# Autodesk Inventor assembly: Ganymede Node
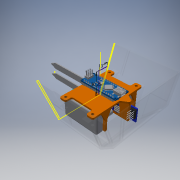
[picture p0: Inventor's stored thumbnail of the model, 180x180]
Saved by Autodesk Inventor 2017 (Build 210142000, 142)
## iProperties
Created: 2017-04-29
Part Number: Ganymede Node
Document SubType Name: Assembly
Designer: X220T
Author: X220T
## Documents named in this file (11)
- C:\Google Drive\Projects\Hackathon\RenoSpaceApps2017\Node Components\Ganymede Node.iam
- C:\Google Drive\Projects\Hackathon\RenoSpaceApps2017\Node Components\NanoV3 v4.ipt
- C:\Google Drive\Projects\Hackathon\RenoSpaceApps2017\Node Components\NRF24L01+.ipt
- C:\Google Drive\Projects\Hackathon\RenoSpaceApps2017\Node Components\solar cell 26x52.ipt
- C:\Google Drive\Projects\Hackathon\RenoSpaceApps2017\Node Components\soil sensor.ipt
- C:\Google Drive\Projects\Hackathon\RenoSpaceApps2017\Node Components\moist probe.ipt
- C:\Google Drive\Projects\Hackathon\RenoSpaceApps2017\Node Components\core printed.ipt
- C:\Google Drive\Projects\Hackathon\RenoSpaceApps2017\Node Components\Step Down voltage regulator LM2596.ipt
- C:\Google Drive\Projects\Hackathon\RenoSpaceApps2017\Node Components\battery.ipt
- C:\Google Drive\Projects\Hackathon\RenoSpaceApps2017\Node Components\Case 1.ipt
- C:\Google Drive\Projects\Hackathon\RenoSpaceApps2017\Node Components\Case 2.ipt
## Components (16 placed, 10 different names)
1. NanoV3 v4:1 — Mate:2, Mate:3, Flush:5
2. NRF24L01+:1 — Mate:6, Flush:6, Mate:7
3. soil sensor:1 — Mate:1, Flush:1, Flush:2
4. moist probe:1 — Mate:1, Flush:1, Flush:2, Flush:3, Mate:2, Mate:3, Mate:4, Flush:4, Mate:5, Flush:5, Mate:6, Flush:6, Mate:7
5. core printed:1 — Flush:3, Rotational:1, Flush:7
6. Step Down voltage regulator LM2596:1 — Rotational:1
7. battery:1
8. battery:2
9. Case 1:1 — Planar:1, Planar:2, Planar:3, Planar:4, Planar:6, Flush:7, Flush:8, Flush:9
10. solar cell 26x52:7
11. solar cell 26x52:9 — Planar:6
12. solar cell 26x52:11 — Planar:3
13. solar cell 26x52:13 — Planar:4
14. solar cell 26x52:15 — Planar:1
15. solar cell 26x52:16 — Planar:2
16. Case 2:1 — Flush:8, Flush:9
## Relationships (22: Flush 9, Mate 7, PlanarJoint 5, RevoluteJoint 1)
- Mate:1 (3.95 mm): soil sensor:1 ↔ moist probe:1
- Flush:1 (-2.68 mm): soil sensor:1 ↔ moist probe:1
- Flush:2: soil sensor:1 ↔ moist probe:1
- Flush:3: moist probe:1 ↔ core printed:1
- Mate:2 (4 mm): NanoV3 v4:1 ↔ moist probe:1
- Mate:3 (-4 mm): NanoV3 v4:1 ↔ moist probe:1
- Mate:4: moist probe:1
- Flush:4: moist probe:1
- Mate:5: moist probe:1
- Flush:5 (9 mm): NanoV3 v4:1 ↔ moist probe:1
- Mate:6 (3 mm): NRF24L01+:1 ↔ moist probe:1
- Flush:6: NRF24L01+:1 ↔ moist probe:1
- Mate:7 (25 mm): NRF24L01+:1 ↔ moist probe:1
- Rotational:1 [RevoluteJoint]: core printed:1 ↔ Step Down voltage regulator LM2596:1
- Planar:1: Case 1:1 ↔ solar cell 26x52:15
- Planar:2: Case 1:1 ↔ solar cell 26x52:16
- Planar:3: Case 1:1 ↔ solar cell 26x52:11
- Planar:4: Case 1:1 ↔ solar cell 26x52:13
- Planar:6: Case 1:1 ↔ solar cell 26x52:9
- Flush:7: core printed:1 ↔ Case 1:1
- Flush:8: Case 1:1 ↔ Case 2:1
- Flush:9: Case 1:1 ↔ Case 2:1
